# Autodesk Inventor assembly: soporte
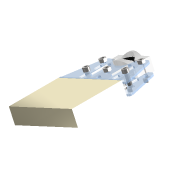
[picture p0: Inventor's stored thumbnail of the model, 180x180]
Saved by Autodesk Inventor 2022 (Build 260153000, 153)
## iProperties
Created: 2022-11-16
Part Number: soporte
Document SubType Name: Assembly
Designer: ferna
Author: ferna
## Documents named in this file (13)
- C:\Users\ferna\Documents\Bocas\Prototipo_09\New folder\soporte.iam
- C:\Users\ferna\Documents\Bocas\Prototipo_09\New folder\soporte_base.ipt
- C:\Users\ferna\Documents\Bocas\Prototipo_09\New folder\soporte_lateral.ipt
- C:\Users\ferna\Documents\Bocas\Prototipo_09\New folder\soporte_medio.ipt
- C:\Users\ferna\Documents\Bocas\Prototipo_08\soporte_flauta_3.ipt
- C:\Users\ferna\Documents\Bocas\Prototipo_08\soporte_flauta_4.ipt
- C:\Users\ferna\Documents\Bocas\Prototipo_09\New folder\goma.ipt
- C:\Users\ferna\Downloads\TeclasFlauta\perno_largo.ipt
- C:\Users\ferna\Documents\Inventor\Content Center Files\R2022\en-US\AS 1112 (2)\AS 1112 - M5  Type 5.ipt
- C:\Users\ferna\Documents\Inventor\Content Center Files\R2022\en-US\ANSI B18.3.1M(1)\ANSI B18.3.1M - M6x1 x 25(2).ipt
- C:\Users\ferna\Documents\Inventor\Content Center Files\R2022\en-US\AS 1112 (2)\AS 1112 - M6  Type 5.ipt
- C:\Users\ferna\Documents\Bocas\Prototipo_09\New folder\base_soportes.ipt
- C:\Users\ferna\Documents\Inventor\Content Center Files\R2022\en-US\AS 1420\AS 1420 - 1973 - M6 x 10.ipt
## Components (26 placed, 12 different names)
1. soporte_base:1 — Mate:1, Mate:2, Mate:3, Mate:4, Mate:5, Mate:6, Mate:7, Mate:8, Mate:9, Mate:10, Mate:11, Mate:12, Angle:1, Mate:38, Mate:39, Mate:40, Mate:43, Mate:44
2. soporte_lateral:1 — Mate:1, Mate:3, Mate:5, Mate:13, Mate:14, Flush:2, Flush:3, Mate:30, Mate:31, Mate:32, Mate:33, Mate:46, Mate:50, Mate:51, Mate:53, Mate:55
3. soporte_medio:1 — Mate:8, Mate:10, Mate:11
4. soporte_lateral:2 — Mate:2, Mate:4, Mate:6, Mate:36, Mate:37, Mate:45, Mate:47, Mate:49, Mate:52, Mate:54, Mate:56
5. soporte_medio:2 — Mate:7, Mate:9, Mate:12
6. soporte_flauta_3:1 — Mate:13, Mate:14, Angle:1, Mate:15, Mate:16, Flush:1, Mate:17, Angle:2, Mate:19, Mate:20, Mate:21, Mate:22, Mate:23, Mate:24
7. soporte_flauta_4:1 — Mate:15, Mate:16, Flush:1, Mate:18, Angle:3, Mate:25, Mate:26, Mate:27, Mate:28
8. goma:1 — Mate:17, Angle:2, Flush:2
9. goma:2 — Mate:18, Angle:3, Flush:3
10. perno_largo:1 — Mate:26, Mate:28
11. perno_largo:2 — Mate:25, Mate:27
12. AS 1112 (2) - Metric M5  Type 5:1 — Mate:22, Mate:23, Mate:24
13. AS 1112 (2) - Metric M5  Type 5:2 — Mate:19, Mate:20, Mate:21
14. Broached Socket Head Cap Screw - Metric M6x1 x 25:1 — Mate:31, Mate:33, Mate:34
15. Broached Socket Head Cap Screw - Metric M6x1 x 25:2 — Mate:30, Mate:32, Mate:35
16. AS 1112 (2) - Metric M6  Type 5:1 — Mate:35, Mate:36
17. AS 1112 (2) - Metric M6  Type 5:2 — Mate:34, Mate:37
18. base_soportes:1 — Mate:38, Mate:39, Mate:40, Mate:41, Mate:42
19. AS 1420 - Metric M6 x 10:1 — Mate:41, Mate:43
20. AS 1420 - Metric M6 x 10:2 — Mate:42, Mate:44
21. AS 1112 (2) - Metric M6  Type 5:3 — Mate:46, Mate:51
22. AS 1112 (2) - Metric M6  Type 5:4 — Mate:45, Mate:54
23. AS 1112 (2) - Metric M6  Type 5:5 — Mate:49, Mate:53
24. AS 1112 (2) - Metric M6  Type 5:6 — Mate:50, Mate:52
25. AS 1112 (2) - Metric M6  Type 5:7 — Mate:48, Mate:55
26. AS 1112 (2) - Metric M6  Type 5:8 — Mate:47, Mate:48, Mate:56
## Relationships (61: Mate 55, Angle 3, Flush 3)
- Mate:1: soporte_base:1 ↔ soporte_lateral:1
- Mate:2: soporte_base:1 ↔ soporte_lateral:2
- Mate:3: soporte_base:1 ↔ soporte_lateral:1
- Mate:4: soporte_base:1 ↔ soporte_lateral:2
- Mate:5: soporte_base:1 ↔ soporte_lateral:1
- Mate:6: soporte_base:1 ↔ soporte_lateral:2
- Mate:7: soporte_base:1 ↔ soporte_medio:2
- Mate:8: soporte_base:1 ↔ soporte_medio:1
- Mate:9: soporte_base:1 ↔ soporte_medio:2
- Mate:10: soporte_base:1 ↔ soporte_medio:1
- Mate:11: soporte_base:1 ↔ soporte_medio:1
- Mate:12: soporte_base:1 ↔ soporte_medio:2
- Mate:13: soporte_lateral:1 ↔ soporte_flauta_3:1
- Mate:14: soporte_lateral:1 ↔ soporte_flauta_3:1
- Angle:1 (180 deg): soporte_base:1 ↔ soporte_flauta_3:1
- Mate:15: soporte_flauta_3:1 ↔ soporte_flauta_4:1
- Mate:16: soporte_flauta_3:1 ↔ soporte_flauta_4:1
- Flush:1 (-15 mm): soporte_flauta_3:1 ↔ soporte_flauta_4:1
- Mate:17: soporte_flauta_3:1 ↔ goma:1
- Angle:2 (30 deg): soporte_flauta_3:1 ↔ goma:1
- Flush:2: soporte_lateral:1 ↔ goma:1
- Mate:18: soporte_flauta_4:1 ↔ goma:2
- Angle:3 (30 deg): soporte_flauta_4:1 ↔ goma:2
- Flush:3: soporte_lateral:1 ↔ goma:2
- Mate:19: soporte_flauta_3:1 ↔ AS 1112 (2) - Metric M5  Type 5:2
- Mate:20 (0.25 mm): soporte_flauta_3:1 ↔ AS 1112 (2) - Metric M5  Type 5:2
- Mate:21 (0.25 mm): soporte_flauta_3:1 ↔ AS 1112 (2) - Metric M5  Type 5:2
- Mate:22: soporte_flauta_3:1 ↔ AS 1112 (2) - Metric M5  Type 5:1
- Mate:23 (0.25 mm): soporte_flauta_3:1 ↔ AS 1112 (2) - Metric M5  Type 5:1
- Mate:24 (0.25 mm): soporte_flauta_3:1 ↔ AS 1112 (2) - Metric M5  Type 5:1
- Mate:25: soporte_flauta_4:1 ↔ perno_largo:2
- Mate:26: soporte_flauta_4:1 ↔ perno_largo:1
- Mate:27: soporte_flauta_4:1 ↔ perno_largo:2
- Mate:28: soporte_flauta_4:1 ↔ perno_largo:1
- Mate:30: soporte_lateral:1 ↔ Broached Socket Head Cap Screw - Metric M6x1 x 25:2
- Mate:31: soporte_lateral:1 ↔ Broached Socket Head Cap Screw - Metric M6x1 x 25:1
- Mate:32: soporte_lateral:1 ↔ Broached Socket Head Cap Screw - Metric M6x1 x 25:2
- Mate:33: soporte_lateral:1 ↔ Broached Socket Head Cap Screw - Metric M6x1 x 25:1
- Mate:34: Broached Socket Head Cap Screw - Metric M6x1 x 25:1 ↔ AS 1112 (2) - Metric M6  Type 5:2
- Mate:35: Broached Socket Head Cap Screw - Metric M6x1 x 25:2 ↔ AS 1112 (2) - Metric M6  Type 5:1
- Mate:36: soporte_lateral:2 ↔ AS 1112 (2) - Metric M6  Type 5:1
- Mate:37: soporte_lateral:2 ↔ AS 1112 (2) - Metric M6  Type 5:2
- Mate:38: soporte_base:1 ↔ base_soportes:1
- Mate:39: soporte_base:1 ↔ base_soportes:1
- Mate:40: soporte_base:1 ↔ base_soportes:1
- Mate:41: base_soportes:1 ↔ AS 1420 - Metric M6 x 10:1
- Mate:42: base_soportes:1 ↔ AS 1420 - Metric M6 x 10:2
- Mate:43: soporte_base:1 ↔ AS 1420 - Metric M6 x 10:1
- Mate:44: soporte_base:1 ↔ AS 1420 - Metric M6 x 10:2
- Mate:45: soporte_lateral:2 ↔ AS 1112 (2) - Metric M6  Type 5:4
- Mate:46: soporte_lateral:1 ↔ AS 1112 (2) - Metric M6  Type 5:3
- Mate:47: soporte_lateral:2 ↔ AS 1112 (2) - Metric M6  Type 5:8
- Mate:48: AS 1112 (2) - Metric M6  Type 5:7 ↔ AS 1112 (2) - Metric M6  Type 5:8
- Mate:49: soporte_lateral:2 ↔ AS 1112 (2) - Metric M6  Type 5:5
- Mate:50: soporte_lateral:1 ↔ AS 1112 (2) - Metric M6  Type 5:6
- Mate:51: soporte_lateral:1 ↔ AS 1112 (2) - Metric M6  Type 5:3
- Mate:52: soporte_lateral:2 ↔ AS 1112 (2) - Metric M6  Type 5:6
- Mate:53: soporte_lateral:1 ↔ AS 1112 (2) - Metric M6  Type 5:5
- Mate:54: soporte_lateral:2 ↔ AS 1112 (2) - Metric M6  Type 5:4
- Mate:55: soporte_lateral:1 ↔ AS 1112 (2) - Metric M6  Type 5:7
- Mate:56: soporte_lateral:2 ↔ AS 1112 (2) - Metric M6  Type 5:8
